# Autodesk Inventor assembly: gehaeuse_bg
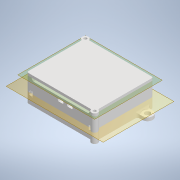
[picture p0: Inventor's stored thumbnail of the model, 180x180]
Saved by Autodesk Inventor 2021.3 (Build 253353010, 353A)
## iProperties
Created: 2021-08-02
Part Number: gehaeuse_bg
Document SubType Name: Assembly
Designer: Markus
Author: Markus
## Documents named in this file (4)
- C:\Users\Markus\Documents\Inventor\MotorController\gehaeuse_bg.iam
- C:\Users\Markus\Documents\Inventor\MotorController\gehause.ipt
- C:\Users\Markus\Documents\Inventor\MotorController\deckel.ipt
- C:\Users\Markus\Documents\Inventor\MotorController\Riegel1.ipt
## Components (3 placed, 3 different names)
1. gehause:1 — Fluchtend:1, Fluchtend:2, Fluchtend:4
2. deckel:1 — Fluchtend:1
3. Riegel1:1 — Fluchtend:3, Fluchtend:4, Fluchtend:5
## Relationships (5: Flush 5)
- Fluchtend:1 [Flush]: gehause:1 ↔ deckel:1
- Fluchtend:2 [Flush] (2.25 mm): gehause:1
- Fluchtend:3 [Flush]: Riegel1:1
- Fluchtend:4 [Flush]: gehause:1 ↔ Riegel1:1
- Fluchtend:5 [Flush]: Riegel1:1
